# Autodesk Inventor assembly: fc17-065
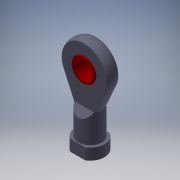
[picture p0: Inventor's stored thumbnail of the model, 180x180]
Saved by Autodesk Inventor 2017.1 (Build 211199000, 199)
## iProperties
Category: Bearings
Company: Autodesk, Inc.
Created: 2016-12-16
Part Number: fc17-065
Catalog Web Link: http://www.igus.com/iPro/iPro_02_0030_0000_USen.htm?ArtNr=EBRI-10R&c=US&l=en
Description: igubal Rod End Bearing
Vendor: igus
Document SubType Name: Assembly
Mass: 29.1846 g
Surface Area: 106.697 cm^2
Volume: 25.0095 cm^3
Density: 1.16694 g/cm^3
Project: FIRST
Designer: Autodesk, Inc.
Title: igubal Rod End Bearing
Author: Autodesk, Inc.
Keywords: FIRST Choice
## Documents named in this file (3)
- D:\FIRST\FIRST KOP 2017\FIRST FirstChoice 2017\fc17-065_RodEnd.iam
- D:\FIRST\FIRST KOP 2017\FIRST FirstChoice 2017\Parts\EBRI-10R_Housing.ipt
- D:\FIRST\FIRST KOP 2017\FIRST FirstChoice 2017\Parts\EBRI-10R_Spherical Bearing.ipt
## Components (2 placed, 2 different names)
1. EBRI-10R_Housing:1 — Mate:1, Angle:1
2. EBRI-10R_Spherical Bearing:1 — Mate:1, Angle:1
## Relationships (2: Mate 1, Angle 1)
- Mate:1: EBRI-10R_Housing:1 ↔ EBRI-10R_Spherical Bearing:1
- Angle:1 (0 deg): EBRI-10R_Housing:1 ↔ EBRI-10R_Spherical Bearing:1
